# Autodesk Inventor assembly: TrackingWheels
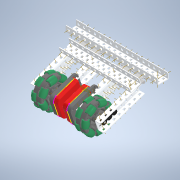
[picture p0: Inventor's stored thumbnail of the model, 180x180]
Saved by Autodesk Inventor 2020 (Build 240168000, 168)
## iProperties
Created: 2019-11-07
Part Number: TrackingWheels
Document SubType Name: Assembly
Designer: Alex Zaccardelli
Author: Alex Zaccardelli
## Documents named in this file (12)
- D:\DR4BTrayBot\ActualCad\TrackingWheels.iam
- D:\DR4BTrayBot\SIGBotsCADLibrary\Structure\C-Channel 2 x 17.ipt
- D:\DR4BTrayBot\SIGBotsCADLibrary\Gussets\Hinge Plate 2.ipt
- D:\DR4BTrayBot\SIGBotsCADLibrary\Gussets\Hinge Pin.ipt
- D:\DR4BTrayBot\SIGBotsCADLibrary\Gussets\Hinge Plate 1.ipt
- D:\DR4BTrayBot\SIGBotsCADLibrary\Motion\Wheel 2.75 inch Omni.ipt
- D:\DR4BTrayBot\SIGBotsCADLibrary\Structure\C-Channel 2 x 13.ipt
- D:\DR4BTrayBot\SIGBotsCADLibrary\Motion\Spacer 0.50 unit.ipt
- D:\DR4BTrayBot\SIGBotsCADLibrary\Structure\C-Channel 2 x 8.ipt
- D:\DR4BTrayBot\SIGBotsCADLibrary\Sensors\Optical Shaft Encoder.iam
- D:\DR4BTrayBot\SIGBotsCADLibrary\Motion\Shaft 3.0 inch.ipt
- D:\DR4BTrayBot\SIGBotsCADLibrary\Motion\Bearing Block.ipt
## Components (26 placed, 11 different names)
1. C-Channel 2 x 17:1
2. Hinge Plate 2:1
3. Hinge Pin:1
4. Hinge Plate 1:1
5. Hinge Plate 2:2
6. Hinge Pin:2
7. Hinge Plate 1:2
8. Wheel Small Omni:1
9. C-Channel 2 x 13:1
10. Spacer 0.50 unit:1
11. Spacer 0.50 unit:2
12. C-Channel 2 x 8:1 — Flush:5, Mate:45, Mate:52, Mate:53, Mate:54
13. C-Channel 2 x 8:2 — Mate:49, Mate:50, Mate:51
14. Optical Shaft Encoder:1 [sub-assembly]
15. Wheel Small Omni:2
16. Spacer 0.50 unit:3
17. Spacer 0.50 unit:4
18. C-Channel 2 x 8:3 — Mate:46, Mate:47, Mate:48
19. C-Channel 2 x 8:4 — Flush:4, Mate:55, Mate:56, Mate:57
20. Optical Shaft Encoder:2 [sub-assembly] — Mate:44
21. Shaft 3.0 inch:1 — Flush:4, Mate:44
22. Shaft 3.0 inch:2 — Flush:5, Mate:45
23. Bearing Block:1 — Mate:46, Mate:47, Mate:48
24. Bearing Block:2 — Mate:49, Mate:50, Mate:51
25. Bearing Block:3 — Mate:52, Mate:53, Mate:54
26. Bearing Block:5 — Mate:55, Mate:56, Mate:57
## Relationships (64: Mate 57, Flush 5, Angle 2)
- [Mate]: C-Channel 2 x 17:1 ↔ Hinge Plate 2:1
- [Mate]: Hinge Pin:1 ↔ Hinge Plate 1:1
- [Mate]: Hinge Plate 2:1 ↔ Hinge Pin:1
- [Flush]: Hinge Pin:1 ↔ Hinge Plate 1:1
- [Mate] (0.381 mm): Hinge Plate 2:1 ↔ Hinge Plate 1:1
- [Mate]: C-Channel 2 x 17:1 ↔ Hinge Plate 2:2
- [Mate]: Hinge Pin:2 ↔ Hinge Plate 1:2
- [Mate]: Hinge Plate 2:2 ↔ Hinge Pin:2
- [Flush]: Hinge Pin:2 ↔ Hinge Plate 1:2
- [Mate] (0.381 mm): Hinge Plate 2:2 ↔ Hinge Plate 1:2
- [Flush]: Hinge Plate 1:1 ↔ Hinge Plate 1:2
- [Mate]: C-Channel 2 x 17:1 ↔ Hinge Plate 2:1
- [Mate]: C-Channel 2 x 17:1 ↔ Hinge Plate 2:1
- [Mate]: C-Channel 2 x 17:1 ↔ Hinge Plate 2:2
- [Mate]: C-Channel 2 x 17:1 ↔ Hinge Plate 2:2
- [Mate]: Hinge Plate 1:1 ↔ C-Channel 2 x 13:1
- [Mate]: Hinge Plate 1:1 ↔ C-Channel 2 x 13:1
- [Mate]: Hinge Plate 1:2 ↔ C-Channel 2 x 13:1
- [Mate]: Wheel Small Omni:1 ↔ Spacer 0.50 unit:1
- [Mate]: Wheel Small Omni:1 ↔ Spacer 0.50 unit:1
- [Mate]: Wheel Small Omni:1 ↔ Spacer 0.50 unit:2
- [Mate]: Wheel Small Omni:1 ↔ Spacer 0.50 unit:2
- [Mate]: Hinge Plate 1:1 ↔ C-Channel 2 x 8:1
- [Mate]: Hinge Plate 1:1 ↔ C-Channel 2 x 8:1
- [Mate]: C-Channel 2 x 13:1 ↔ C-Channel 2 x 8:1
- [Mate] (6.5278 mm): Wheel Small Omni:1 ↔ C-Channel 2 x 8:1
- [Mate]: Hinge Plate 1:1 ↔ C-Channel 2 x 8:2
- [Mate]: C-Channel 2 x 13:1 ↔ C-Channel 2 x 8:2
- [Mate]: C-Channel 2 x 13:1 ↔ C-Channel 2 x 8:2
- [Mate]: Spacer 0.50 unit:1 ↔ C-Channel 2 x 8:1
- [Mate] (6.35 mm): C-Channel 2 x 8:2 ↔ Optical Shaft Encoder:1
- [Mate]: Spacer 0.50 unit:2 ↔ Optical Shaft Encoder:1
- [Angle] (0 deg): C-Channel 2 x 8:2 ↔ Optical Shaft Encoder:1
- [Mate]: Wheel Small Omni:2 ↔ Spacer 0.50 unit:3
- [Mate]: Wheel Small Omni:2 ↔ Spacer 0.50 unit:3
- [Mate]: Wheel Small Omni:2 ↔ Spacer 0.50 unit:4
- [Mate]: Wheel Small Omni:2 ↔ Spacer 0.50 unit:4
- [Mate] (6.5278 mm): Wheel Small Omni:2 ↔ C-Channel 2 x 8:3
- [Mate]: Spacer 0.50 unit:3 ↔ C-Channel 2 x 8:3
- [Mate]: Hinge Plate 1:2 ↔ C-Channel 2 x 8:4
- [Mate]: Hinge Plate 1:2 ↔ C-Channel 2 x 8:4
- [Mate]: C-Channel 2 x 13:1 ↔ C-Channel 2 x 8:4
- [Mate]: Hinge Plate 1:2 ↔ C-Channel 2 x 8:3
- [Mate]: C-Channel 2 x 13:1 ↔ C-Channel 2 x 8:3
- [Mate]: C-Channel 2 x 13:1 ↔ C-Channel 2 x 8:3
- [Mate] (6.35 mm): C-Channel 2 x 8:3 ↔ Optical Shaft Encoder:2
- [Mate]: C-Channel 2 x 8:3 ↔ Optical Shaft Encoder:2
- [Angle] (0 deg): C-Channel 2 x 8:3 ↔ Optical Shaft Encoder:2
- Flush:4 (5.08 mm): C-Channel 2 x 8:4 ↔ Shaft 3.0 inch:1
- Mate:44: Optical Shaft Encoder:2 ↔ Shaft 3.0 inch:1
- Flush:5 (5.08 mm): C-Channel 2 x 8:1 ↔ Shaft 3.0 inch:2
- Mate:45: C-Channel 2 x 8:1 ↔ Shaft 3.0 inch:2
- Mate:46: C-Channel 2 x 8:3 ↔ Bearing Block:1
- Mate:47: C-Channel 2 x 8:3 ↔ Bearing Block:1
- Mate:48: C-Channel 2 x 8:3 ↔ Bearing Block:1
- Mate:49: C-Channel 2 x 8:2 ↔ Bearing Block:2
- Mate:50: C-Channel 2 x 8:2 ↔ Bearing Block:2
- Mate:51: C-Channel 2 x 8:2 ↔ Bearing Block:2
- Mate:52: C-Channel 2 x 8:1 ↔ Bearing Block:3
- Mate:53: C-Channel 2 x 8:1 ↔ Bearing Block:3
- Mate:54: C-Channel 2 x 8:1 ↔ Bearing Block:3
- Mate:55: C-Channel 2 x 8:4 ↔ Bearing Block:5
- Mate:56: C-Channel 2 x 8:4 ↔ Bearing Block:5
- Mate:57: C-Channel 2 x 8:4 ↔ Bearing Block:5
## Named parameters: d360_d342 = 0 mm, d361_d343 = 0 mm, d362_d344 = 0 mm, d363_d345 = 0 mm, d364_d352 = 6.5278 mm, d365_d356 = 0 mm, d307_d2 = 0 mm, d308_d3 = 0.381 mm, d312_d0 = 0 mm, d313_d1 = 0 mm, d314_d2 = 0 mm, d315_d3 = 0.381 mm
